# Autodesk Inventor assembly: pasekturbonowy
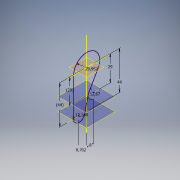
[picture p0: Inventor's stored thumbnail of the model, 180x180]
Saved by Autodesk Inventor 2019 (Build 230136000, 136)
## iProperties
Created: 2020-08-27
Part Number: pasekturbonowy
Document SubType Name: Assembly
Designer: estee
Author: estee
## Documents named in this file (3)
- C:\Users\estee\OneDrive\Pulpit\estere\1\MUM\nowygit\Mechanika\Moduł obrotu RET Estera\projejt\pasekturbonowy.iam
- C:\Users\estee\OneDrive\Pulpit\estere\1\MUM\nowygit\Mechanika\Moduł obrotu RET Estera\projejt\czesc1paska.ipt
- C:\Users\estee\OneDrive\Pulpit\estere\1\MUM\nowygit\Mechanika\Moduł obrotu RET Estera\projejt\zab.ipt
## Components (2 placed, 2 different names)
1. czesc1paska:1 — Flush:1, Flush:2, Flush:3, Mate:1, Mate:2, Mate:3
2. zab:1 — Mate:3
## Relationships (6: Flush 3, Mate 3)
- Flush:1: czesc1paska:1
- Flush:2: czesc1paska:1
- Flush:3: czesc1paska:1
- Mate:1 (-44 mm): czesc1paska:1
- Mate:2 (-29 mm): czesc1paska:1
- Mate:3: czesc1paska:1 ↔ zab:1
